# Autodesk Inventor assembly: Kit Frame 24x32
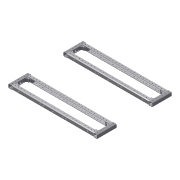
[picture p0: Inventor's stored thumbnail of the model, 180x180]
Saved by Autodesk Inventor 2013 (Build 170138000, 138)
## iProperties
Created: 2013-01-06
Part Number: Kit Frame 24x32
Document SubType Name: Assembly
Designer: Nemo
Author: Nemo
## Documents named in this file (4)
- \\lmss\STUDENTS\Robotics\CAD Files\COTS Parts\Kit Frame - AndyMark\Kit Frame 24x32.iam
- \\lmss\STUDENTS\Robotics\CAD Files\COTS Parts\Kit Frame - AndyMark\Components\24x34 Side Rail sub.iam
- \\lmss\STUDENTS\Robotics\CAD Files\COTS Parts\Kit Frame - AndyMark\Components\24x32 Side Rail Sub mirror.iam
- C:\Users\dagulick\robotics\.625 kit frame.ipt
## Components (8 placed, 3 different names)
1. 24x34 Side Rail sub:1 [sub-assembly] — Flush:11, Flush:12, Mate:6, Flush:13, Flush:14
2. 24x34 Side Rail sub:2 [sub-assembly] — Flush:4, Flush:7, Mate:5, Flush:8, Mate:7
3. 24x32 Side Rail Sub mirror:1 [sub-assembly] — Flush:3, Mate:3, Flush:16, Flush:17
4. 24x32 Side Rail Sub mirror:2 [sub-assembly] — Flush:5, Flush:6, Mate:4, Flush:11, Flush:12, Flush:15
5. .625 kit frame:1 — Flush:3, Flush:4, Mate:3, Mate:7
6. .625 kit frame:2 — Flush:5, Flush:6, Mate:4
7. .625 kit frame:3 — Mate:6, Flush:13, Flush:14, Flush:15
8. .625 kit frame:4 — Flush:7, Mate:5, Flush:8, Flush:16, Flush:17
## Relationships (22: Flush 15, Mate 7)
- [Mate] (36.83 mm): 24x34 Side Rail sub:1
- [Flush]: 24x34 Side Rail sub:1 ↔ 24x32 Side Rail Sub mirror:1
- [Mate]: 24x34 Side Rail sub:1
- [Flush]: 24x32 Side Rail Sub mirror:1
- Flush:3: 24x32 Side Rail Sub mirror:1 ↔ .625 kit frame:1
- Flush:4: 24x34 Side Rail sub:2 ↔ .625 kit frame:1
- Mate:3: 24x32 Side Rail Sub mirror:1 ↔ .625 kit frame:1
- Flush:5: 24x32 Side Rail Sub mirror:2 ↔ .625 kit frame:2
- Flush:6: 24x32 Side Rail Sub mirror:2 ↔ .625 kit frame:2
- Mate:4: 24x32 Side Rail Sub mirror:2 ↔ .625 kit frame:2
- Flush:7: 24x34 Side Rail sub:2 ↔ .625 kit frame:4
- Mate:5: 24x34 Side Rail sub:2 ↔ .625 kit frame:4
- Flush:8: 24x34 Side Rail sub:2 ↔ .625 kit frame:4
- Flush:11: 24x34 Side Rail sub:1 ↔ 24x32 Side Rail Sub mirror:2
- Flush:12: 24x34 Side Rail sub:1 ↔ 24x32 Side Rail Sub mirror:2
- Mate:6: 24x34 Side Rail sub:1 ↔ .625 kit frame:3
- Flush:13: 24x34 Side Rail sub:1 ↔ .625 kit frame:3
- Flush:14: 24x34 Side Rail sub:1 ↔ .625 kit frame:3
- Flush:15: 24x32 Side Rail Sub mirror:2 ↔ .625 kit frame:3
- Flush:16: 24x32 Side Rail Sub mirror:1 ↔ .625 kit frame:4
- Flush:17: 24x32 Side Rail Sub mirror:1 ↔ .625 kit frame:4
- Mate:7: 24x34 Side Rail sub:2 ↔ .625 kit frame:1
